# Autodesk Inventor assembly: MVFKN40
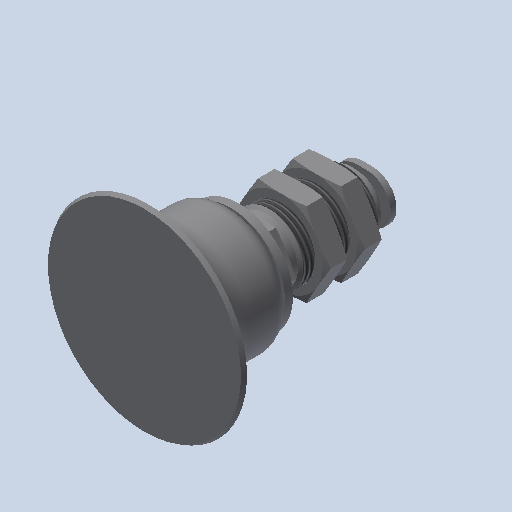
[picture p0: Inventor's stored thumbnail of the model, 512x512]
Saved by Autodesk Inventor 2024.1 (Build 281209000, 209)
## iProperties
Created: 2023-12-16
Part Number: MVFKN40
Catalog Web Link: www.cadenas.de
Description: MVPKN, MVPKE, MVPKF, MVFKN, MVFKF-Suction Cups - Standard Type - Standard / Deep
Vendor: MISUMI
Document SubType Name: Assembly
Designer: psAdmin
Manufacturer: MISUMI
Mass: 15.5291 g
Surface Area: 64.8522 cm^2
Volume: 15.5291 cm^3
Density: 1 g/cm^3
Category: PARTsolutions
Company: MISUMI
PSOL_IDENT_0: {$CADENAS_DATA/23d-libs/misumi/metric/35_tubes_nozzles/mvpke_asmtab.prj},195 {VTYP=3D},{STYP=ASSTAB}
PSOL_IDENT_1: ,{NB=MVFKN40},{LINA=MVFKN40},{NN=MVPKN, MVPKE, MVPKF, MVFKN, MVFKF},{DATE=04.06.2021 06:55:05},{GEOM
PSOL_IDENT_2: DATE=07.07.2014},{VERSION=},{LINEID=20},{WBVAR=MATP,NO},{WBNUMERIC=NO}  {NB=MVFKN40},{LINA=MVFKN40},
PSOL_IDENT_3: {KT=DUMMY},{PN=MVFKN40},{MATM=Brass},{TYPE=MVFKN},{ST=Electroless Nickel Plating},{SHAPE=Deep},{MATP=
PSOL_IDENT_4: N},{MATPALG='N', 'Nitrile Rubber','F','Fluoro Rubber'},{AC=Suction Cup (VPFT)},{NO=40},{NOALG=20,25,
PSOL_IDENT_5: 30,40},{D=6},{DD=40},{L1=17.5},{B=45.2},{L2=23.1},{L3=18.0},{H1=17},{T=4},{M=M14x1.0},{MASS=47.0},{T
PSOL_IDENT_6: IFF=2},{MVPNT=1},{MVPFT=1},{PPATH=mvpkn/mvpkn_asmtpl.prj},{MVPKN=1}
NB: MVFKN40
NN: MVPKN, MVPKE, MVPKF, MVFKN, MVFKF
NT: Suction Cups - Standard Type - Standard / Deep
NBSYN: $PN.
LINA: MVFKN40
CATALOG: Misumi
PN: MVFKN40
SHAPE: Deep
MATP: Nitrile Rubber
AC: Suction Cup (VPFT)
NO: 40
D: 6
DD: 40
L1: 17.5
B: 45.2
L2: 23.1
L3: 18
H1: 17
T: 4
M: M14x1.0
MASS: 47
SUPPLIER: MISUMI
ARTICLENO: MVFKN40
BOMINFO: MVFKN40
CREATOR: CADENAS GmbH
Title: MVFKN40
Author: Cadenas PARTsolutions
Comments: Suction Cups - Standard Type - Standard / Deep
## Documents named in this file (3)
- C:\Users\haruy\OneDrive - Kyushu University\KURT_工房共有\2023~2024\ハード\CAD\2024NHK\000_parts\吸着パッド\MVFKN40_Autodesk_Inventor_2024_20231216\AIS2024\MVFKN40.iam
- C:\Users\haruy\OneDrive - Kyushu University\KURT_工房共有\2023~2024\ハード\CAD\2024NHK\000_parts\吸着パッド\MVFKN40_Autodesk_Inventor_2024_20231216\AIS2024\MVFKN40-1-1.ipt
- C:\Users\haruy\OneDrive - Kyushu University\KURT_工房共有\2023~2024\ハード\CAD\2024NHK\000_parts\吸着パッド\MVFKN40_Autodesk_Inventor_2024_20231216\AIS2024\MVFKN40-NUT-NUT.ipt
## Components (3 placed, 2 different names)
1. MVFKN40-1-1:1 — body_to_nut3_Z@1 <-> NUT_TO_BODY_Z@2, body_to_nut4_Z@1 <-> NUT_TO_BODY_Z@3
2. MVFKN40-NUT-NUT:1 — body_to_nut3_Z@1 <-> NUT_TO_BODY_Z@2
3. MVFKN40-NUT-NUT:2 — body_to_nut4_Z@1 <-> NUT_TO_BODY_Z@3
## Relationships (2: Mate 2)
- body_to_nut3_Z@1 <-> NUT_TO_BODY_Z@2 [Mate]: MVFKN40-1-1:1 ↔ MVFKN40-NUT-NUT:1
- body_to_nut4_Z@1 <-> NUT_TO_BODY_Z@3 [Mate]: MVFKN40-1-1:1 ↔ MVFKN40-NUT-NUT:2
